# Autodesk Inventor assembly: Wine Glass Rack Full Assembly
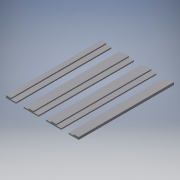
[picture p0: Inventor's stored thumbnail of the model, 180x180]
Saved by Autodesk Inventor 2016 (Build 200138000, 138)
## iProperties
Created: 2017-10-31
Part Number: Wine Glass Rack Full Assembly
Document SubType Name: Assembly
Designer: mathaetaes
Author: mathaetaes
## Documents named in this file (3)
- E:\Projects\3D Printer\printer projects\My Designs\Bar Cabinet 2.2.2018\Wine Glass Rack Full Assembly.iam
- E:\Projects\3D Printer\printer projects\My Designs\Bar Cabinet 2.2.2018\Wine Glass Rack Edge.iam
- E:\Projects\3D Printer\printer projects\My Designs\Bar Cabinet 2.2.2018\Wine Glass Rack Middle.iam
## Components (4 placed, 2 different names)
1. Wine Glass Rack Edge:1 [sub-assembly] — Flush:1, Flush:4, Mate:3
2. Wine Glass Rack Edge:2 [sub-assembly] — Flush:3, Flush:6, Mate:1
3. Wine Glass Rack Middle:1 [sub-assembly] — Flush:1, Flush:2, Flush:4, Flush:5, Mate:2, Mate:3, Mate:4
4. Wine Glass Rack Middle:2 [sub-assembly] — Flush:2, Flush:3, Flush:5, Flush:6, Mate:1, Mate:2, Mate:4
## Relationships (10: Flush 6, Mate 4)
- Flush:1: Wine Glass Rack Edge:1 ↔ Wine Glass Rack Middle:1
- Flush:2: Wine Glass Rack Middle:1 ↔ Wine Glass Rack Middle:2
- Flush:3: Wine Glass Rack Edge:2 ↔ Wine Glass Rack Middle:2
- Flush:4: Wine Glass Rack Edge:1 ↔ Wine Glass Rack Middle:1
- Flush:5: Wine Glass Rack Middle:1 ↔ Wine Glass Rack Middle:2
- Flush:6: Wine Glass Rack Edge:2 ↔ Wine Glass Rack Middle:2
- Mate:1 (38.1 mm): Wine Glass Rack Edge:2 ↔ Wine Glass Rack Middle:2
- Mate:2 (38.1 mm): Wine Glass Rack Middle:1 ↔ Wine Glass Rack Middle:2
- Mate:3 (38.1 mm): Wine Glass Rack Edge:1 ↔ Wine Glass Rack Middle:1
- Mate:4 (38.1 mm): Wine Glass Rack Middle:1 ↔ Wine Glass Rack Middle:2
## Named parameters: StemWidth = 38.1 mm
